# Autodesk Inventor assembly: Bearing_Belt_Assembly
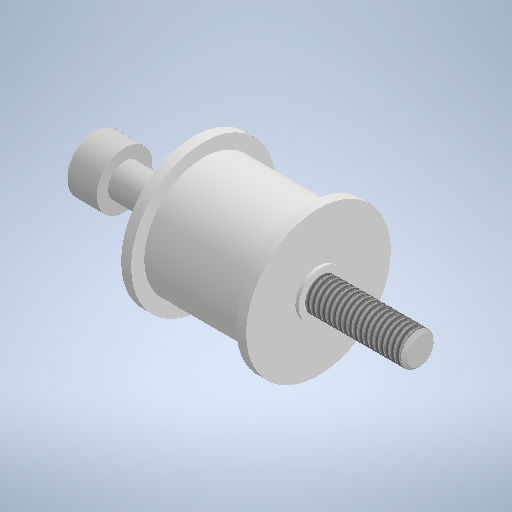
[picture p0: Inventor's stored thumbnail of the model, 512x512]
Saved by Autodesk Inventor 2025.1 (Build 291241020, 241B)
## iProperties
Created: 2024-11-07
Part Number: Bearing_Belt_Assembly
Document SubType Name: Assembly
Designer: leon-
Author: leon-
## Documents named in this file (5)
- C:\Users\leon-\OneDrive\Dokumente\Education\Berkeley\Embedded_Systems\Project\CAD Model\Bearing_Belt_Assembly.iam
- C:\Users\leon-\OneDrive\Dokumente\Education\Berkeley\Embedded_Systems\Project\CAD Model\Purchase_Parts\Belt_Bearing.ipt
- Belt_Bearing_5M12T_16_5.ipt
- C:\Users\leon-\OneDrive\Dokumente\Education\Berkeley\Embedded_Systems\Project\CAD Model\Bearing_Belt_Distance_Sleeve.ipt
- C:\Users\leon-\OneDrive\Dokumente\Education\Berkeley\Embedded_Systems\Project\CAD Model\Purchase_Parts\SCB5-45.ipt
## Components (4 placed, 3 different names)
1. Belt_Bearing_5M12T_16_5:1 — Mate:1, Mate:2, Mate:3, Mate:4
2. Bearing_Belt_Distance_Sleeve:1 — Mate:2, Mate:3, Mate:5, Mate:6
3. Bearing_Belt_Distance_Sleeve:2 — Mate:1, Mate:4
4. SCB5-45:1 — Mate:5, Mate:6
## Relationships (6: Mate 6)
- Mate:1: Belt_Bearing_5M12T_16_5:1 ↔ Bearing_Belt_Distance_Sleeve:2
- Mate:2: Belt_Bearing_5M12T_16_5:1 ↔ Bearing_Belt_Distance_Sleeve:1
- Mate:3: Belt_Bearing_5M12T_16_5:1 ↔ Bearing_Belt_Distance_Sleeve:1
- Mate:4: Belt_Bearing_5M12T_16_5:1 ↔ Bearing_Belt_Distance_Sleeve:2
- Mate:5: Bearing_Belt_Distance_Sleeve:1 ↔ SCB5-45:1
- Mate:6 (10 mm): Bearing_Belt_Distance_Sleeve:1 ↔ SCB5-45:1
